# Autodesk Inventor assembly: Assembly1
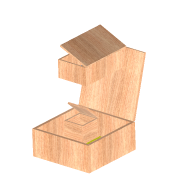
[picture p0: Inventor's stored thumbnail of the model, 180x180]
Saved by Autodesk Inventor 2020.2 (Build 242310000, 310)
## iProperties
Created: 2020-02-23
Part Number: Assembly1
Document SubType Name: Assembly
Designer: Svend
Author: Svend
## Documents named in this file (12)
- C:\Users\Svend\OneDrive\Documents\Inventor\VerjaardagJuul\Assembly1.iam
- C:\Users\Svend\OneDrive\Documents\Inventor\VerjaardagJuul\onderEnBovenplaat.ipt
- C:\Users\Svend\OneDrive\Documents\Inventor\VerjaardagJuul\zijkant.ipt
- C:\Users\Svend\OneDrive\Documents\Inventor\VerjaardagJuul\bovenplaat.ipt
- C:\Users\Svend\OneDrive\Documents\Inventor\VerjaardagJuul\lp.ipt
- C:\Users\Svend\OneDrive\Documents\Inventor\VerjaardagJuul\bodemKleineDoos.ipt
- C:\Users\Svend\OneDrive\Documents\Inventor\VerjaardagJuul\zijkantKleineDoos.ipt
- C:\Users\Svend\OneDrive\Documents\Inventor\VerjaardagJuul\bovenkantKleineDoos.ipt
- C:\Users\Svend\OneDrive\Documents\Inventor\VerjaardagJuul\onderkantMiddenDoos.ipt
- C:\Users\Svend\OneDrive\Documents\Inventor\VerjaardagJuul\zijkantMiddenDoos.ipt
- C:\Users\Svend\OneDrive\Documents\Inventor\VerjaardagJuul\zijkant2MiddenDoos.ipt
- C:\Users\Svend\OneDrive\Documents\Inventor\VerjaardagJuul\bovenkantMiddenDoos.ipt
## Components (19 placed, 11 different names)
1. onderEnBovenplaat:1 — Mate:1, Flush:1, Flush:2, Mate:2, Flush:4, Flush:5, Mate:4, Mate:5, Flush:7, Mate:8
2. zijkant:1 — Mate:1, Flush:1, Flush:2, Flush:3, Mate:6, Flush:8, Mate:10, Mate:17
3. zijkant:2 — Mate:2, Flush:3, Flush:4, Flush:6, Mate:7, Mate:18, Mate:26
4. zijkant:3 — Flush:5, Mate:4, Flush:6, Mate:27
5. zijkant:4 — Mate:5, Mate:6, Flush:7, Mate:9
6. bovenplaat:1 — Mate:7, Flush:8
7. lp:1 — Mate:8, Mate:9, Mate:10, Mate:16
8. bodemKleineDoos:1 — Flush:9, Mate:11, Flush:10, Flush:11, Flush:13, Mate:14, Flush:15, Mate:16
9. zijkantKleineDoos:1 — Flush:11, Mate:12, Flush:12, Mate:13, Flush:14, Mate:17, Flush:16
10. zijkantKleineDoos:2 — Flush:13, Mate:13, Flush:14, Mate:15, Mate:18, Mate:19
11. zijkantKleineDoos:3 — Mate:14, Mate:15, Flush:15
12. zijkantKleineDoos:4 — Flush:9, Mate:11, Flush:10, Mate:12, Flush:12
13. bovenkantKleineDoos:1 — Mate:19, Flush:16
14. onderkantMiddenDoos:1 — Flush:17, Mate:20, Flush:18, Mate:21, Flush:19, Flush:20, Mate:22, Flush:21, Mate:24, Flush:22
15. zijkantMiddenDoos:1 — Flush:17, Mate:20, Flush:18, Mate:25, Flush:23
16. zijkantMiddenDoos:2 — Mate:21, Flush:19, Flush:20, Mate:23, Mate:26
17. zijkant2MiddenDoos:1 — Mate:22, Flush:21, Mate:23
18. zijkant2MiddenDoos:2 — Mate:24, Flush:22, Mate:25, Mate:27, Mate:28
19. bovenkantMiddenDoos:1 — Mate:28, Flush:23
## Relationships (50: Mate 27, Flush 23)
- Mate:1: onderEnBovenplaat:1 ↔ zijkant:1
- Flush:1: onderEnBovenplaat:1 ↔ zijkant:1
- Flush:2: onderEnBovenplaat:1 ↔ zijkant:1
- Mate:2: onderEnBovenplaat:1 ↔ zijkant:2
- Flush:3: zijkant:1 ↔ zijkant:2
- Flush:4: onderEnBovenplaat:1 ↔ zijkant:2
- Flush:5: onderEnBovenplaat:1 ↔ zijkant:3
- Mate:4: onderEnBovenplaat:1 ↔ zijkant:3
- Flush:6: zijkant:2 ↔ zijkant:3
- Mate:5: onderEnBovenplaat:1 ↔ zijkant:4
- Mate:6: zijkant:1 ↔ zijkant:4
- Flush:7: onderEnBovenplaat:1 ↔ zijkant:4
- Mate:7: zijkant:2 ↔ bovenplaat:1
- Flush:8: zijkant:1 ↔ bovenplaat:1
- Mate:8: onderEnBovenplaat:1 ↔ lp:1
- Mate:9 (7.5 mm): zijkant:4 ↔ lp:1
- Mate:10 (7.5 mm): zijkant:1 ↔ lp:1
- Flush:9: bodemKleineDoos:1 ↔ zijkantKleineDoos:4
- Mate:11: bodemKleineDoos:1 ↔ zijkantKleineDoos:4
- Flush:10: bodemKleineDoos:1 ↔ zijkantKleineDoos:4
- Flush:11: bodemKleineDoos:1 ↔ zijkantKleineDoos:1
- Mate:12: zijkantKleineDoos:1 ↔ zijkantKleineDoos:4
- Flush:12: zijkantKleineDoos:1 ↔ zijkantKleineDoos:4
- Flush:13: bodemKleineDoos:1 ↔ zijkantKleineDoos:2
- Mate:13: zijkantKleineDoos:1 ↔ zijkantKleineDoos:2
- Flush:14: zijkantKleineDoos:1 ↔ zijkantKleineDoos:2
- Mate:14: bodemKleineDoos:1 ↔ zijkantKleineDoos:3
- Mate:15: zijkantKleineDoos:2 ↔ zijkantKleineDoos:3
- Flush:15: bodemKleineDoos:1 ↔ zijkantKleineDoos:3
- Mate:16: lp:1 ↔ bodemKleineDoos:1
- Mate:17 (15 mm): zijkant:1 ↔ zijkantKleineDoos:1
- Mate:18 (15 mm): zijkant:2 ↔ zijkantKleineDoos:2
- Mate:19: zijkantKleineDoos:2 ↔ bovenkantKleineDoos:1
- Flush:16: zijkantKleineDoos:1 ↔ bovenkantKleineDoos:1
- Flush:17: onderkantMiddenDoos:1 ↔ zijkantMiddenDoos:1
- Mate:20: onderkantMiddenDoos:1 ↔ zijkantMiddenDoos:1
- Flush:18: onderkantMiddenDoos:1 ↔ zijkantMiddenDoos:1
- Mate:21: onderkantMiddenDoos:1 ↔ zijkantMiddenDoos:2
- Flush:19: onderkantMiddenDoos:1 ↔ zijkantMiddenDoos:2
- Flush:20: onderkantMiddenDoos:1 ↔ zijkantMiddenDoos:2
- Mate:22: onderkantMiddenDoos:1 ↔ zijkant2MiddenDoos:1
- Flush:21: onderkantMiddenDoos:1 ↔ zijkant2MiddenDoos:1
- Mate:23: zijkantMiddenDoos:2 ↔ zijkant2MiddenDoos:1
- Mate:24: onderkantMiddenDoos:1 ↔ zijkant2MiddenDoos:2
- Flush:22: onderkantMiddenDoos:1 ↔ zijkant2MiddenDoos:2
- Mate:25: zijkantMiddenDoos:1 ↔ zijkant2MiddenDoos:2
- Mate:26 (7.5 mm): zijkant:2 ↔ zijkantMiddenDoos:2
- Mate:27 (7.5 mm): zijkant:3 ↔ zijkant2MiddenDoos:2
- Mate:28: zijkant2MiddenDoos:2 ↔ bovenkantMiddenDoos:1
- Flush:23: zijkantMiddenDoos:1 ↔ bovenkantMiddenDoos:1
